# Autodesk Inventor assembly: bumper test
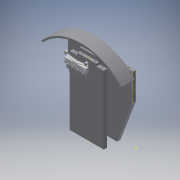
[picture p0: Inventor's stored thumbnail of the model, 180x180]
Saved by Autodesk Inventor 2016 (Build 200138000, 138)
## iProperties
Created: 2015-09-30
Part Number: bumper test
Document SubType Name: Assembly
Designer: Jesse Stevenson
Author: Jesse Stevenson
## Documents named in this file (7)
- C:\Users\Jesse Stevenson\Desktop\robot\bumper test.iam
- C:\Users\Jesse Stevenson\Desktop\robot\top.ipt
- C:\Users\Jesse Stevenson\Desktop\robot\bottom.ipt
- C:\Users\Jesse Stevenson\Desktop\robot\Microswitch_-_Omron_D2SW-P2L2T.iam
- C:\Users\Jesse Stevenson\Desktop\robot\bumper lever support.ipt
- C:\Users\Jesse Stevenson\Desktop\robot\lever2.ipt
- C:\Users\Jesse Stevenson\Desktop\robot\bumper.ipt
## Components (8 placed, 6 different names)
1. top:1 — Flush:1, Mate:1, Mate:2, Angle:2
2. bottom:1 — Flush:1, Mate:1, Mate:3, Mate:5, Mate:6, Flush:3, Flush:4
3. Microswitch_-_Omron_D2SW-P2L2T:1 [sub-assembly] — Mate:5, Mate:7, Flush:2
4. Microswitch_-_Omron_D2SW-P2L2T:2 [sub-assembly] — Mate:6, Mate:7, Flush:2
5. bumper lever support:1 — Flush:3, Flush:4, Mate:8, Mate:9, Mate:10, Mate:11
6. lever2:1 — Mate:8, Mate:9, Mate:16
7. lever2:2 — Mate:10, Mate:11, Mate:14, Mate:15
8. bumper:1 — Angle:2, Mate:13, Mate:14, Mate:15, Mate:16
## Relationships (20: Mate 15, Flush 4, Angle 1)
- Flush:1: top:1 ↔ bottom:1
- Mate:1 (18.923 mm): top:1 ↔ bottom:1
- Mate:2: top:1
- Mate:3: bottom:1
- Mate:4 (25.273 mm)
- Mate:5 (12.7 mm): bottom:1 ↔ Microswitch_-_Omron_D2SW-P2L2T:1
- Mate:6 (12.7 mm): bottom:1 ↔ Microswitch_-_Omron_D2SW-P2L2T:2
- Mate:7: Microswitch_-_Omron_D2SW-P2L2T:1 ↔ Microswitch_-_Omron_D2SW-P2L2T:2
- Flush:2: Microswitch_-_Omron_D2SW-P2L2T:1 ↔ Microswitch_-_Omron_D2SW-P2L2T:2
- Flush:3: bottom:1 ↔ bumper lever support:1
- Flush:4: bottom:1 ↔ bumper lever support:1
- Mate:8: bumper lever support:1 ↔ lever2:1
- Mate:9: bumper lever support:1 ↔ lever2:1
- Mate:10: bumper lever support:1 ↔ lever2:2
- Mate:11: bumper lever support:1 ↔ lever2:2
- Angle:2 (180 deg): top:1 ↔ bumper:1
- Mate:13: bumper:1
- Mate:14: lever2:2 ↔ bumper:1
- Mate:15: lever2:2 ↔ bumper:1
- Mate:16: lever2:1 ↔ bumper:1
